# Autodesk Inventor assembly: 5933 robot
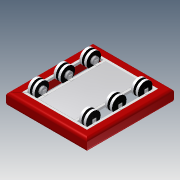
[picture p0: Inventor's stored thumbnail of the model, 180x180]
Saved by Autodesk Inventor 2014 (Build 180170000, 170)
## iProperties
Created: 2016-01-12
Part Number: 5933 robot
Document SubType Name: Assembly
Designer: Paul
Mass: 47071.7 g
Surface Area: 36225.8 cm^2
Volume: 40090.2 cm^3
Density: 1.17414 g/cm^3
Author: Paul
## Documents named in this file (11)
- C:\Users\Paul\Documents\Inventor\first 2016\5933 robot.iam
- C:\Users\Paul\Documents\Inventor\first 2016\frame side rail.ipt
- C:\Users\Paul\Documents\Inventor\first 2016\frame inside rail.ipt
- C:\Users\Paul\Documents\Inventor\first 2016\frame end rail.ipt
- C:\Users\Paul\Documents\Inventor\first 2016\axlesupport end.ipt
- C:\Users\Paul\Documents\Inventor\first 2016\wheeldblsprocket.iam
- C:\Users\Paul\Documents\Inventor\first 2016\axlesupport center.ipt
- C:\Users\Paul\Documents\Inventor\first 2016\bumper side.ipt
- C:\Users\Paul\Documents\Inventor\first 2016\bumper front.ipt
- C:\Users\Paul\Documents\Inventor\first 2016\375x5bolt.ipt
- C:\Users\Paul\Documents\Inventor\first 2016\base plate.ipt
## Components (35 placed, 10 different names)
1. frame side rail:1 — Flush:1, Flush:2, Flush:3, Mate:1, Mate:3, Mate:4, Mate:6, Flush:6, Flush:7, Mate:9, Mate:10, Flush:23, Mate:32, Mate:44, Flush:27
2. frame side rail:2 — Flush:3, Mate:2, Mate:5, Flush:4, Flush:5, Mate:7, Mate:8, Flush:12, Mate:15, Mate:25, Mate:26, Flush:19, Mate:27
3. frame inside rail:1 — Flush:21, Mate:34, Flush:24, Mate:35, Flush:25, Flush:26, Mate:43, Mate:49
4. frame inside rail:2 — Mate:19, Mate:20, Mate:21, Flush:15, Flush:16, Flush:17, Flush:18, Mate:50, Mate:64
5. frame end rail:1 — Flush:1, Mate:1, Mate:2, Mate:4, Flush:8, Flush:11, Flush:17, Mate:25, Flush:22, Mate:30, Mate:65
6. frame end rail:2 — Flush:2, Mate:3, Mate:5, Mate:6, Flush:9, Flush:10, Flush:13, Mate:28, Flush:20, Flush:21, Mate:49, Mate:50
7. axlesupport end:1 — Flush:7, Mate:10, Flush:9, Mate:36, Mate:38, Mate:60
8. axlesupport end:2 — Flush:6, Mate:9, Flush:8, Mate:37, Mate:39, Mate:61, Mate:62
9. axlesupport end:3 — Flush:4, Mate:7, Flush:11, Mate:11, Mate:12, Mate:55, Mate:56
10. axlesupport end:4 — Flush:5, Mate:8, Flush:10, Mate:14, Mate:18, Mate:52
11. wheeldblsprocket:1 [sub-assembly] — Mate:11, Mate:12, Mate:23
12. wheeldblsprocket:7 [sub-assembly] — Mate:14, Mate:18, Mate:22, Mate:51
13. axlesupport center:1 — Flush:12, Mate:15, Mate:16, Mate:17, Flush:13, Mate:54
14. wheeldblsprocket:3 [sub-assembly] — Mate:16, Mate:17, Mate:24, Mate:48
15. axlesupport end:5 — Mate:19, Flush:15, Mate:22
16. axlesupport end:6 — Mate:21, Flush:16, Mate:23
17. axlesupport center:2 — Mate:20, Flush:18, Mate:24, Mate:53
18. bumper side:1 — Mate:26, Flush:19, Mate:27, Mate:29, Mate:31
19. bumper front:1 — Mate:28, Flush:20, Mate:29
20. bumper front:2 — Flush:22, Mate:30, Mate:31, Mate:33
21. bumper side:2 — Flush:23, Mate:32, Mate:33
22. axlesupport end:7 — Mate:34, Flush:24, Mate:41, Mate:59, Mate:63
23. axlesupport end:8 — Mate:35, Flush:25, Mate:40, Mate:42
24. wheeldblsprocket:4 [sub-assembly] — Mate:36, Mate:38, Mate:41
25. wheeldblsprocket:5 [sub-assembly] — Mate:45, Mate:46, Mate:47, Mate:48
26. wheeldblsprocket:6 [sub-assembly] — Mate:37, Mate:39, Mate:40, Mate:42
27. axlesupport center:3 — Flush:26, Mate:43, Mate:46
28. axlesupport center:4 — Mate:44, Flush:27, Mate:45, Mate:47, Mate:57, Mate:58
29. 375x5bolt:1 — Mate:51, Mate:52
30. 375x5bolt:2 — Mate:55, Mate:56
31. 375x5bolt:3 — Mate:53, Mate:54
32. 375x5bolt:4 — Mate:59, Mate:60
33. 375x5bolt:5 — Mate:57, Mate:58
34. 375x5bolt:6 — Mate:61, Mate:62
35. base plate:1 — Mate:63, Mate:64, Mate:65
## Relationships (90: Mate 64, Flush 26)
- Flush:1: frame side rail:1 ↔ frame end rail:1
- Flush:2: frame side rail:1 ↔ frame end rail:2
- Flush:3: frame side rail:1 ↔ frame side rail:2
- Mate:1: frame side rail:1 ↔ frame end rail:1
- Mate:2: frame side rail:2 ↔ frame end rail:1
- Mate:3: frame side rail:1 ↔ frame end rail:2
- Mate:4: frame side rail:1 ↔ frame end rail:1
- Mate:5: frame side rail:2 ↔ frame end rail:2
- Mate:6: frame side rail:1 ↔ frame end rail:2
- Flush:4: frame side rail:2 ↔ axlesupport end:3
- Flush:5: frame side rail:2 ↔ axlesupport end:4
- Flush:6: frame side rail:1 ↔ axlesupport end:2
- Flush:7: frame side rail:1 ↔ axlesupport end:1
- Mate:7: frame side rail:2 ↔ axlesupport end:3
- Mate:8: frame side rail:2 ↔ axlesupport end:4
- Mate:9: frame side rail:1 ↔ axlesupport end:2
- Mate:10: frame side rail:1 ↔ axlesupport end:1
- Flush:8 (82.55 mm): frame end rail:1 ↔ axlesupport end:2
- Flush:9 (-82.55 mm): frame end rail:2 ↔ axlesupport end:1
- Flush:10 (-82.55 mm): frame end rail:2 ↔ axlesupport end:4
- Flush:11 (-82.55 mm): frame end rail:1 ↔ axlesupport end:3
- Mate:11: axlesupport end:3 ↔ wheeldblsprocket:1
- Mate:12 (4.7625 mm): axlesupport end:3 ↔ wheeldblsprocket:1
- Mate:14 (4.7625 mm): axlesupport end:4 ↔ wheeldblsprocket:7
- Flush:12: frame side rail:2 ↔ axlesupport center:1
- Mate:15: frame side rail:2 ↔ axlesupport center:1
- Mate:16: axlesupport center:1 ↔ wheeldblsprocket:3
- Mate:17 (4.7625 mm): axlesupport center:1 ↔ wheeldblsprocket:3
- Flush:13 (-355.6 mm): frame end rail:2 ↔ axlesupport center:1
- Mate:18: axlesupport end:4 ↔ wheeldblsprocket:7
- Mate:19: frame inside rail:2 ↔ axlesupport end:5
- Mate:20: frame inside rail:2 ↔ axlesupport center:2
- Mate:21: frame inside rail:2 ↔ axlesupport end:6
- Flush:15: frame inside rail:2 ↔ axlesupport end:5
- Flush:16: frame inside rail:2 ↔ axlesupport end:6
- Mate:22: wheeldblsprocket:7 ↔ axlesupport end:5
- Flush:17: frame inside rail:2 ↔ frame end rail:1
- Mate:23 (4.7625 mm): wheeldblsprocket:1 ↔ axlesupport end:6
- Flush:18: frame inside rail:2 ↔ axlesupport center:2
- Mate:24: wheeldblsprocket:3 ↔ axlesupport center:2
- Mate:25: frame side rail:2 ↔ frame end rail:1
- Mate:26: frame side rail:2 ↔ bumper side:1
- Flush:19: frame side rail:2 ↔ bumper side:1
- Mate:27: frame side rail:2 ↔ bumper side:1
- Mate:28: frame end rail:2 ↔ bumper front:1
- Flush:20: frame end rail:2 ↔ bumper front:1
- Mate:29: bumper side:1 ↔ bumper front:1
- Flush:21: frame inside rail:1 ↔ frame end rail:2
- Flush:22: frame end rail:1 ↔ bumper front:2
- Mate:30: frame end rail:1 ↔ bumper front:2
- Mate:31: bumper side:1 ↔ bumper front:2
- Flush:23: frame side rail:1 ↔ bumper side:2
- Mate:32: frame side rail:1 ↔ bumper side:2
- Mate:33: bumper front:2 ↔ bumper side:2
- Mate:34: frame inside rail:1 ↔ axlesupport end:7
- Flush:24: frame inside rail:1 ↔ axlesupport end:7
- Mate:35: frame inside rail:1 ↔ axlesupport end:8
- Flush:25: frame inside rail:1 ↔ axlesupport end:8
- Mate:36: axlesupport end:1 ↔ wheeldblsprocket:4
- Mate:37: axlesupport end:2 ↔ wheeldblsprocket:6
- Mate:38 (4.7625 mm): axlesupport end:1 ↔ wheeldblsprocket:4
- Mate:39 (4.7625 mm): axlesupport end:2 ↔ wheeldblsprocket:6
- Mate:40: axlesupport end:8 ↔ wheeldblsprocket:6
- Mate:41: axlesupport end:7 ↔ wheeldblsprocket:4
- Mate:42 (4.7625 mm): axlesupport end:8 ↔ wheeldblsprocket:6
- Flush:26: frame inside rail:1 ↔ axlesupport center:3
- Mate:43: frame inside rail:1 ↔ axlesupport center:3
- Mate:44: frame side rail:1 ↔ axlesupport center:4
- Flush:27: frame side rail:1 ↔ axlesupport center:4
- Mate:45 (4.7625 mm): wheeldblsprocket:5 ↔ axlesupport center:4
- Mate:46: wheeldblsprocket:5 ↔ axlesupport center:3
- Mate:47: wheeldblsprocket:5 ↔ axlesupport center:4
- Mate:48: wheeldblsprocket:3 ↔ wheeldblsprocket:5
- Mate:49: frame inside rail:1 ↔ frame end rail:2
- Mate:50: frame inside rail:2 ↔ frame end rail:2
- Mate:51: wheeldblsprocket:7 ↔ 375x5bolt:1
- Mate:52: axlesupport end:4 ↔ 375x5bolt:1
- Mate:53: axlesupport center:2 ↔ 375x5bolt:3
- Mate:54: axlesupport center:1 ↔ 375x5bolt:3
- Mate:55: axlesupport end:3 ↔ 375x5bolt:2
- Mate:56: axlesupport end:3 ↔ 375x5bolt:2
- Mate:57: axlesupport center:4 ↔ 375x5bolt:5
- Mate:58: axlesupport center:4 ↔ 375x5bolt:5
- Mate:59: axlesupport end:7 ↔ 375x5bolt:4
- Mate:60: axlesupport end:1 ↔ 375x5bolt:4
- Mate:61: axlesupport end:2 ↔ 375x5bolt:6
- Mate:62: axlesupport end:2 ↔ 375x5bolt:6
- Mate:63: axlesupport end:7 ↔ base plate:1
- Mate:64: frame inside rail:2 ↔ base plate:1
- Mate:65: frame end rail:1 ↔ base plate:1
